# Autodesk Inventor assembly: LAP RAP KHOP NOI MEM
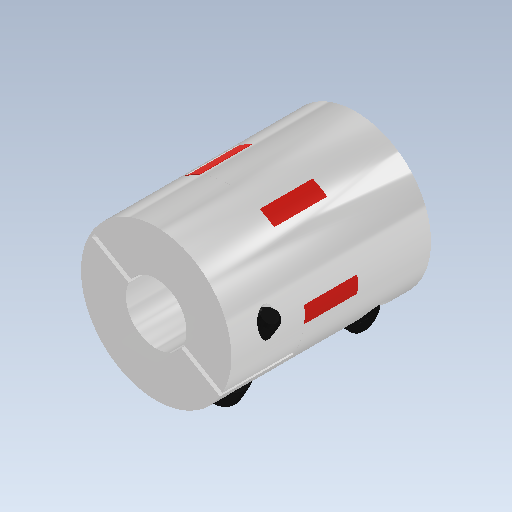
[picture p0: Inventor's stored thumbnail of the model, 512x512]
Saved by Autodesk Inventor 2021 (Build 250183000, 183)
## iProperties
Created: 2022-03-09
Part Number: LAP RAP KHOP NOI MEM
Document SubType Name: Assembly
Designer: 41601100
Author: 41601100
## Documents named in this file (5)
- C:\Users\authe\OneDrive\Desktop\Gripper7Inv\LAP RAP KHOP NOI MEM.iam
- C:\Users\authe\OneDrive\Desktop\Gripper7Inv\PHAN NHOM 6.ipt
- C:\Users\authe\OneDrive\Desktop\Gripper7Inv\PHAN NHOM.ipt
- C:\Users\authe\OneDrive\Desktop\Gripper7Inv\LUC GIAC.ipt
- C:\Users\authe\OneDrive\Desktop\Gripper7Inv\CAO SU KHOP.ipt
## Components (5 placed, 4 different names)
1. PHAN NHOM 6:1 — Mate:1, Mate:3, Mate:5, Mate:6, Mate:7, Mate:8, Mate:10
2. PHAN NHOM:1 — Mate:1, Mate:2, Mate:4, Mate:9, Mate:10
3. LUC GIAC:1 — Mate:2, Mate:4
4. LUC GIAC:2 — Mate:3, Mate:5
5. CAO SU KHOP:1 — Mate:6, Mate:7, Mate:8, Mate:9
## Relationships (10: Mate 10)
- Mate:1: PHAN NHOM 6:1 ↔ PHAN NHOM:1
- Mate:2: PHAN NHOM:1 ↔ LUC GIAC:1
- Mate:3: PHAN NHOM 6:1 ↔ LUC GIAC:2
- Mate:4: PHAN NHOM:1 ↔ LUC GIAC:1
- Mate:5: PHAN NHOM 6:1 ↔ LUC GIAC:2
- Mate:6: PHAN NHOM 6:1 ↔ CAO SU KHOP:1
- Mate:7: PHAN NHOM 6:1 ↔ CAO SU KHOP:1
- Mate:8: PHAN NHOM 6:1 ↔ CAO SU KHOP:1
- Mate:9: PHAN NHOM:1 ↔ CAO SU KHOP:1
- Mate:10: PHAN NHOM 6:1 ↔ PHAN NHOM:1
